# Autodesk Inventor assembly: Ball Transfer Unit Assembly
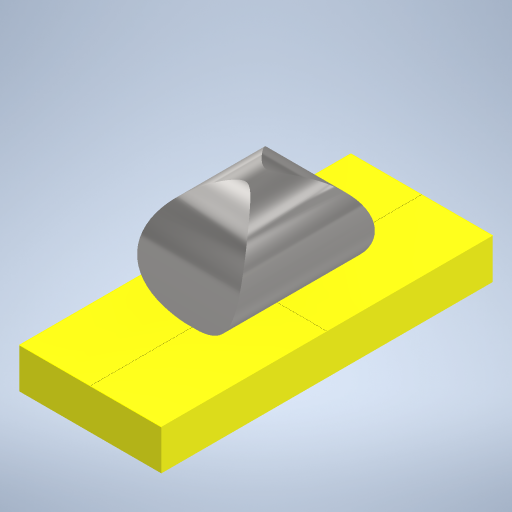
[picture p0: Inventor's stored thumbnail of the model, 512x512]
Saved by Autodesk Inventor 2023 (Build 270158000, 158)
## iProperties
Created: 2022-12-06
Part Number: Ball Transfer Unit Assembly
Document SubType Name: Assembly
Designer: mihal
Mass: 95.6773 g
Surface Area: 82.7763 cm^2
Volume: 27.0206 cm^3
Density: 3.54091 g/cm^3
Author: mihal
## Documents named in this file (3)
- C:\Users\mihal\Documents\Ball Transfer Unit Assembly.iam
- C:\Users\mihal\Desktop\4th Year Project\BHSS DESIGN\Sixth Assembly\ball transfer unit.ipt
- C:\Users\mihal\Desktop\4th Year Project\BHSS DESIGN\Sixth Assembly\ball transfer unit base.ipt
## Components (2 placed, 2 different names)
1. ball transfer unit:1 — Mate:1, Mate:2, Mate:3
2. ball transfer unit base:1 — Mate:1, Mate:2, Mate:3
## Relationships (3: Mate 3)
- Mate:1: ball transfer unit:1 ↔ ball transfer unit base:1
- Mate:2: ball transfer unit:1 ↔ ball transfer unit base:1
- Mate:3: ball transfer unit:1 ↔ ball transfer unit base:1
